# Autodesk Inventor assembly: Assembly1
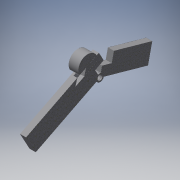
[picture p0: Inventor's stored thumbnail of the model, 180x180]
Saved by Autodesk Inventor 2019 (Build 230136000, 136)
## iProperties
Created: 2018-07-06
Part Number: Assembly1
Document SubType Name: Assembly
Designer: HIVE
Author: HIVE
## Documents named in this file (4)
- D:\hive\projects\knee-patella\Assembly1.iam
- D:\hive\projects\knee-patella\knee ball.ipt
- D:\hive\projects\knee-patella\lower leg.ipt
- D:\hive\projects\knee-patella\upper leg.ipt
## Components (3 placed, 3 different names)
1. knee ball:1 — Mate:6, Mate:7
2. lower leg:1 — Mate:4, Mate:5, Mate:6, Mate:7
3. upper leg:1 — Mate:4, Mate:5
## Relationships (4: Mate 4)
- Mate:4: lower leg:1 ↔ upper leg:1
- Mate:5 (0.2 mm): lower leg:1 ↔ upper leg:1
- Mate:6: knee ball:1 ↔ lower leg:1
- Mate:7: knee ball:1 ↔ lower leg:1
## Named parameters: kneeBallBaseW = 30 mm, kneeBallBaseL = 30 mm, kneeBallBaseH = 10 mm, legDiam = 40 mm, clearance = 0.2 mm
